# Autodesk Inventor assembly: Lower Arm-N
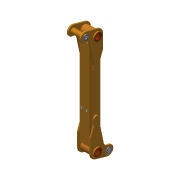
[picture p0: Inventor's stored thumbnail of the model, 180x180]
Saved by Autodesk Inventor 2022 Beta2 (Build 260130000, 130) ContinuousBuild 0
## iProperties
Shininess: 64.0
Length Units: 11269
Angle Units: 11279
Time Units: 11290
Mass Units: 11283
Length Display Precision: 3
Angle Display Precision: 2
Compacted: True
Created: 2003-04-13
Part Number: Lower Arm-N
Document SubType Name: Assembly
Designer: Uffe Bak
Density: 0.0
Volumn: 0.0
Area: 0.0
PropertySet Name: Model Information
Control State: 0
Master: False
Checked Out: False
Author: Uffe Bak
## Documents named in this file (6)
- C:\Autodesk Inventor 2021 Intro Practice Files\BOM\Lower Arm-N.iam
- C:\Autodesk Inventor 2021 Intro Practice Files\BOM\3136 7044 74.ipt
- C:\Autodesk Inventor 2021 Intro Practice Files\BOM\3136 7044 79.ipt
- C:\Autodesk Inventor 2021 Intro Practice Files\BOM\3136 7057 14.ipt
- C:\Autodesk Inventor 2021 Intro Practice Files\BOM\0147 1323 03.ipt
- C:\Autodesk Inventor 2021 Intro Practice Files\BOM\3136 1144 16-N.iam
## Components (13 placed, 5 different names)
1. 3136 7044 74:1 — Mate:1, Flush:1, Insert:1, Insert:3
2. 3136 7044 79:1 — Insert:1, Insert:2
3. 3136 7057 14:1 — Insert:2
4. 0147 1323 03:1
5. 3136 7044 74:2 — Insert:5, Insert:6, Insert:8
6. 3136 1144 16-N:1 [sub-assembly] — Mate:1, Flush:1, Insert:5
7. 3136 7044 79:2 — Insert:3, Insert:4
8. 3136 7057 14:2 — Insert:4
9. 3136 7044 79:3 — Insert:8, Insert:9
10. 3136 7057 14:3 — Insert:9
11. 3136 7044 79:4 — Insert:6, Insert:7
12. 3136 7057 14:4 — Insert:7
13. 0147 1323 03:2
## Relationships (11: Insert 9, Mate 1, Flush 1)
- Mate:1: 3136 7044 74:1 ↔ 3136 1144 16-N:1
- Flush:1 (2.25 mm): 3136 7044 74:1 ↔ 3136 1144 16-N:1
- Insert:1: 3136 7044 74:1 ↔ 3136 7044 79:1
- Insert:2: 3136 7044 79:1 ↔ 3136 7057 14:1
- Insert:3: 3136 7044 74:1 ↔ 3136 7044 79:2
- Insert:4: 3136 7044 79:2 ↔ 3136 7057 14:2
- Insert:5 (-2.25 mm): 3136 7044 74:2 ↔ 3136 1144 16-N:1
- Insert:6: 3136 7044 74:2 ↔ 3136 7044 79:4
- Insert:7: 3136 7044 79:4 ↔ 3136 7057 14:4
- Insert:8: 3136 7044 74:2 ↔ 3136 7044 79:3
- Insert:9: 3136 7044 79:3 ↔ 3136 7057 14:3
